# Autodesk Inventor assembly: fc18-051
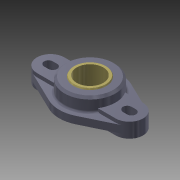
[picture p0: Inventor's stored thumbnail of the model, 180x180]
Saved by Autodesk Inventor 2018 (Build 220112000, 112)
## iProperties
Created: 2017-11-23
Part Number: fc18-051
Description: STEP AP214
Document SubType Name: Assembly
Designer: PhillipD
Preprocessor: Spatial InterOp 3D
Title: EFOI_16_1.stp
Author: igus GmbH
## Documents named in this file (3)
- F:\FIRST 2018\FIRST 2018 FirstChoice\fc18-051.iam
- F:\FIRST 2018\FIRST 2018 FirstChoice\Parts\2017_11_23__19-45-43-821.ipt
- F:\FIRST 2018\FIRST 2018 FirstChoice\Parts\2017_11_23__19-45-43-821_1.ipt
## Components (2 placed, 2 different names)
1. 2017_11_23__19-45-43-821 — Ball:1
2. 2017_11_23__19-45-43-821_1 — Ball:1
## Relationships (1: BallJoint 1)
- Ball:1: 2017_11_23__19-45-43-821 ↔ 2017_11_23__19-45-43-821_1
